# Autodesk Inventor assembly: Diff_test
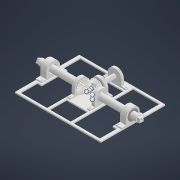
[picture p0: Inventor's stored thumbnail of the model, 180x180]
Saved by Autodesk Inventor 2021 (Build 250183000, 183)
## iProperties
Created: 2021-01-24
Part Number: Diff_test
Document SubType Name: Assembly
Designer: Ctroi
Author: Ctroi
## Documents named in this file (12)
- G:\Roverprojekt\Github Projekt\Rover\Diff_test.iam
- G:\Roverprojekt\Github Projekt\Rover\Testplatte_Differential.ipt
- G:\Roverprojekt\Github Projekt\Rover\Halterung_Differential.ipt
- G:\Roverprojekt\Github Projekt\Rover\Kugellager.ipt
- G:\Roverprojekt\Github Projekt\Rover\Halterung_Differential_2.ipt
- G:\Roverprojekt\Github Projekt\Rover\Verbindung_Rocker_Body.ipt
- G:\Roverprojekt\Github Projekt\Rover\Kegelrad.ipt
- G:\Roverprojekt\Github Projekt\Rover\Halterung_Differential_Mitte.ipt
- G:\Roverprojekt\Github Projekt\Rover\Kugellager_klein.ipt
- G:\Roverprojekt\Github Projekt\Rover\Welle_Kugellager_Mitte.ipt
- G:\Roverprojekt\Github Projekt\Rover\Gegenstück_Welle_Diff.ipt
- G:\Roverprojekt\Github Projekt\Rover\Halterung_Differential_3.ipt
## Components (20 placed, 11 different names)
1. Testplatte_Differential:1 — Passend:5, Passend:6, Passend:7, Passend:8, Passend:9, Passend:10, Passend:39, Passend:40, Passend:41, Passend:48, Passend:49, Passend:50, Passend:51, Passend:52, Passend:53
2. Kugellager:1 — Passend:54, Passend:55
3. Halterung_Differential:1 — Passend:8, Passend:9, Passend:10, Passend:13, Passend:14, Passend:16, Passend:17
4. Halterung_Differential:2 — Passend:5, Passend:6, Passend:7, Passend:11, Passend:12, Passend:15
5. Kugellager:3 — Passend:11, Passend:12, Passend:25, Passend:26
6. Kugellager:4 — Passend:13, Passend:14, Passend:20, Passend:21
7. Halterung_Differential_2:1 — Passend:15, Passend:16, Passend:17, Passend:18, Passend:19
8. Kugellager:5 — Passend:18, Passend:19, Passend:44, Passend:45
9. Verbindung_Rocker_Body:1 — Passend:20, Passend:21, Passend:22, Passend:23, Passend:24
10. Kegelrad2:1 — Passend:22, Passend:23, Passend:24
11. Kegelrad2:2 — Passend:46
12. Verbindung_Rocker_Body:2 — Passend:25, Passend:26, Passend:27, Passend:28
13. Kegelrad2:3 — Passend:27, Passend:28
14. Halterung_Differential_Mitte:1 — Passend:39, Passend:40, Passend:41, Passend:42, Passend:43
15. Kugellager_klein:1 — Passend:42, Passend:43
16. Welle_Kugellager_Mitte:1 — Passend:44, Passend:45, Passend:46, Passend:47
17. Gegenstück_Welle_Diff:1 — Passend:47
18. Halterung_Differential_3:1 — Passend:48, Passend:49, Passend:50, Passend:54, Passend:55
19. Halterung_Differential_3:2 — Passend:51, Passend:52, Passend:53, Passend:56, Passend:57
20. Kugellager:6 — Passend:56, Passend:57
## Relationships (43: Mate 43)
- Passend:5 [Mate]: Testplatte_Differential:1 ↔ Halterung_Differential:2
- Passend:6 [Mate]: Testplatte_Differential:1 ↔ Halterung_Differential:2
- Passend:7 [Mate]: Testplatte_Differential:1 ↔ Halterung_Differential:2
- Passend:8 [Mate]: Testplatte_Differential:1 ↔ Halterung_Differential:1
- Passend:9 [Mate]: Testplatte_Differential:1 ↔ Halterung_Differential:1
- Passend:10 [Mate]: Testplatte_Differential:1 ↔ Halterung_Differential:1
- Passend:11 [Mate]: Halterung_Differential:2 ↔ Kugellager:3
- Passend:12 [Mate]: Halterung_Differential:2 ↔ Kugellager:3
- Passend:13 [Mate]: Halterung_Differential:1 ↔ Kugellager:4
- Passend:14 [Mate]: Halterung_Differential:1 ↔ Kugellager:4
- Passend:15 [Mate]: Halterung_Differential:2 ↔ Halterung_Differential_2:1
- Passend:16 [Mate]: Halterung_Differential:1 ↔ Halterung_Differential_2:1
- Passend:17 [Mate]: Halterung_Differential:1 ↔ Halterung_Differential_2:1
- Passend:18 [Mate]: Halterung_Differential_2:1 ↔ Kugellager:5
- Passend:19 [Mate]: Halterung_Differential_2:1 ↔ Kugellager:5
- Passend:20 [Mate]: Kugellager:4 ↔ Verbindung_Rocker_Body:1
- Passend:21 [Mate]: Kugellager:4 ↔ Verbindung_Rocker_Body:1
- Passend:22 [Mate]: Verbindung_Rocker_Body:1 ↔ Kegelrad2:1
- Passend:23 [Mate]: Verbindung_Rocker_Body:1 ↔ Kegelrad2:1
- Passend:24 [Mate]: Verbindung_Rocker_Body:1 ↔ Kegelrad2:1
- Passend:25 [Mate]: Kugellager:3 ↔ Verbindung_Rocker_Body:2
- Passend:26 [Mate]: Kugellager:3 ↔ Verbindung_Rocker_Body:2
- Passend:27 [Mate]: Verbindung_Rocker_Body:2 ↔ Kegelrad2:3
- Passend:28 [Mate]: Verbindung_Rocker_Body:2 ↔ Kegelrad2:3
- Passend:39 [Mate]: Testplatte_Differential:1 ↔ Halterung_Differential_Mitte:1
- Passend:40 [Mate]: Testplatte_Differential:1 ↔ Halterung_Differential_Mitte:1
- Passend:41 [Mate]: Testplatte_Differential:1 ↔ Halterung_Differential_Mitte:1
- Passend:42 [Mate]: Halterung_Differential_Mitte:1 ↔ Kugellager_klein:1
- Passend:43 [Mate]: Halterung_Differential_Mitte:1 ↔ Kugellager_klein:1
- Passend:44 [Mate]: Kugellager:5 ↔ Welle_Kugellager_Mitte:1
- Passend:45 [Mate]: Kugellager:5 ↔ Welle_Kugellager_Mitte:1
- Passend:46 [Mate]: Kegelrad2:2 ↔ Welle_Kugellager_Mitte:1
- Passend:47 [Mate]: Welle_Kugellager_Mitte:1 ↔ Gegenstück_Welle_Diff:1
- Passend:48 [Mate]: Testplatte_Differential:1 ↔ Halterung_Differential_3:1
- Passend:49 [Mate]: Testplatte_Differential:1 ↔ Halterung_Differential_3:1
- Passend:50 [Mate]: Testplatte_Differential:1 ↔ Halterung_Differential_3:1
- Passend:51 [Mate]: Testplatte_Differential:1 ↔ Halterung_Differential_3:2
- Passend:52 [Mate]: Testplatte_Differential:1 ↔ Halterung_Differential_3:2
- Passend:53 [Mate]: Testplatte_Differential:1 ↔ Halterung_Differential_3:2
- Passend:54 [Mate]: Kugellager:1 ↔ Halterung_Differential_3:1
- Passend:55 [Mate]: Kugellager:1 ↔ Halterung_Differential_3:1
- Passend:56 [Mate]: Halterung_Differential_3:2 ↔ Kugellager:6
- Passend:57 [Mate]: Halterung_Differential_3:2 ↔ Kugellager:6
